# Autodesk Inventor assembly: ASY PRS 9800 DrainSystemBottom_D1200
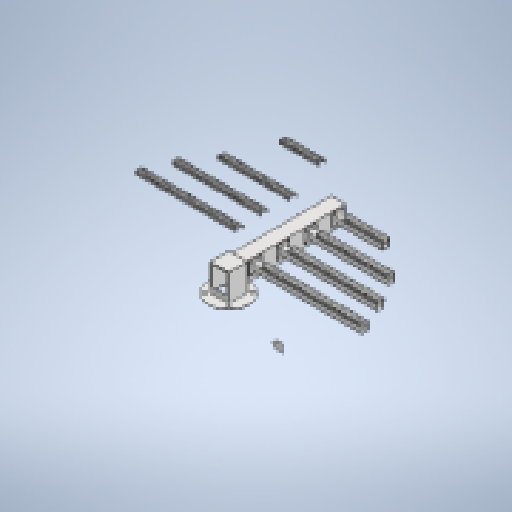
[picture p0: Inventor's stored thumbnail of the model, 512x512]
Saved by Autodesk Inventor 2026.2 (Build 302298000, 298)
## iProperties
Created: 2026-05-12
Part Number: ASY PRS 9800 DrainSystemBottom_D1200
Document SubType Name: Assembly
Designer: admin
Author: admin
## Documents named in this file (22)
- C:\Users\admin\Documents\Inventor\PRS-Purovsk\ASY PRS 9800 DrainSystemBottom_D1200.iam
- C:\Users\admin\Documents\Inventor\PRS-Purovsk\PRS 9651 DrSysB MAIN  FLANGE_D1200.ipt
- C:\Users\admin\Documents\Inventor\PRS-Purovsk\PRS 1425 DrSysB Way FLANGE_D1200.ipt
- C:\Users\admin\Documents\Inventor\PRS-Purovsk\PRS 1401 DrSysB DIMentions_D1200.ipt
- C:\Users\admin\Documents\Inventor\PRS-Purovsk\PRS 1662 DrSysB way tube 4_D1200.ipt
- C:\Users\admin\Documents\Inventor\PRS-Purovsk\PRS 1652 DrSysB Central tube wall_D1200.ipt
- C:\Users\admin\Documents\Inventor\PRS-Purovsk\PRS 1662 DrSysB way tube 2_D1200.ipt
- C:\Users\admin\Documents\Inventor\PRS-Purovsk\PRS 1665 DrSysB CUP 1_D1200.ipt
- C:\Users\admin\Documents\Inventor\PRS-Purovsk\PRS-1666 FDS 1000 CUP 1_D1200.ipt
- C:\Users\admin\Documents\Inventor\PRS-Purovsk\PRS 1422 DrSysB diameter way up_D1200.ipt
- C:\Users\admin\Documents\Inventor\PRS-Purovsk\PRS 1423 DrSysB diameter way down_D1200.ipt
- C:\Users\admin\Documents\Inventor\PRS-Purovsk\PRS 1424 DrSysB diam way cup_D1200.ipt
- C:\Users\admin\Documents\Inventor\PRS-Purovsk\PRS 1661 DrSysB way tube 1_D1200.ipt
- C:\Users\admin\Documents\Inventor\PRS-Purovsk\PRS 5311 DrSysB roof 1_D1200.ipt
- C:\Users\admin\Documents\Inventor\PRS-Purovsk\PRS 5321 DrSysB roof 2_D1200.ipt
- C:\Users\admin\Documents\Inventor\PRS-Purovsk\PRS 5333 DrSysB roof 3_D1200.ipt
- C:\Users\admin\Documents\Inventor\PRS-Purovsk\PRS 1662 DrSysB way tube 44_D1200.ipt
- C:\Users\admin\Documents\Inventor\PRS-Purovsk\PRS 5335 DrSysB roof 33_D1200.ipt
- C:\Users\admin\Documents\Inventor\PRS-Purovsk\PRS 7623 DrSysB  roof 1_1200x7.5_D1200.ipt
- C:\Users\admin\Documents\Inventor\PRS-Purovsk\PRS 5322 DrSysB roof 2_1200x7.5_D1200.ipt
- C:\Users\admin\Documents\Inventor\PRS-Purovsk\PRS 5334 DrSysB roof 3_1200x7.5_D1200.ipt
- C:\Users\admin\Documents\Inventor\PRS-Purovsk\PRS 5336 DrSysB roof 3_44_1200x7.5_D1200.ipt
## Components (28 placed, 21 different names)
1. PRS 9651 DrSysB MAIN  FLANGE_D1200:1 — Flush:8, Flush:7, Mate:3
2. PRS 1425 DrSysB Way FLANGE_D1200:1 — Rigid:4, Rigid:19
3. PRS 1401 DrSysB DIMentions_D1200:1
4. PRS 1662 DrSysB way tube 4_D1200:1 — Flush:5, Mate:9, Mate:7, Rigid:21
5. PRS 1652 DrSysB Central tube wall_D1200:1 — Flush:8, Flush:7, Mate:10, Rigid:24, Rigid:22
6. PRS 1652 DrSysB Central tube wall_D1200:2 — Mate:3, Rigid:22
7. PRS 1662 DrSysB way tube 2_D1200:1 — Mate:8, Flush:6, Mate:6, Rigid:20
8. PRS 1665 DrSysB CUP 1_D1200:1 — Mate:10
9. PRS-1666 FDS 1000 CUP 1_D1200:1
10. PRS 1422 DrSysB diameter way up_D1200:1 — Flush:10, Flush:9, Mate:11, Rigid:23, Rigid:18, Rigid:17, Rigid:16
11. PRS 1423 DrSysB diameter way down_D1200:1 — Rigid:24, Rigid:23, Rigid:4, Rigid:14, Rigid:15, Rigid:13
12. PRS 1424 DrSysB diam way cup_D1200:1 — Flush:10, Flush:9, Mate:11
13. PRS 1425 DrSysB Way FLANGE_D1200:2 — Rigid:20, Rigid:14
14. PRS 1425 DrSysB Way FLANGE_D1200:3 — Rigid:21, Rigid:15
15. PRS 1425 DrSysB Way FLANGE_D1200:4 — Rigid:18
16. PRS 1425 DrSysB Way FLANGE_D1200:5 — Rigid:17
17. PRS 1425 DrSysB Way FLANGE_D1200:6 — Rigid:16
18. PRS 1661 DrSysB way tube 1_D1200:1 — Mate:5, Mate:4, Flush:4, Rigid:19
19. PRS 5311 DrSysB roof 1_D1200:1 — Mate:5, Mate:4, Flush:4
20. PRS 5321 DrSysB roof 2_D1200:1 — Mate:8, Flush:6, Mate:6
21. PRS 5333 DrSysB roof 3_D1200:1 — Flush:5, Mate:9, Mate:7
22. PRS 1662 DrSysB way tube 44_D1200:1 — Mate:12, Mate:13, Flush:9, Rigid:14
23. PRS 5335 DrSysB roof 33_D1200:1 — Mate:12, Mate:13, Flush:9
24. PRS 1425 DrSysB Way FLANGE_D1200:7 — Rigid:13, Rigid:14
25. PRS 7623 DrSysB  roof 1_1200x7.5_D1200:1
26. PRS 5322 DrSysB roof 2_1200x7.5_D1200:1
27. PRS 5334 DrSysB roof 3_1200x7.5_D1200:1
28. PRS 5336 DrSysB roof 3_44_1200x7.5_D1200:1
## Relationships (33: WeldJoint 14, Mate 11, Flush 8)
- Flush:8: PRS 9651 DrSysB MAIN  FLANGE_D1200:1 ↔ PRS 1652 DrSysB Central tube wall_D1200:1
- Flush:7: PRS 9651 DrSysB MAIN  FLANGE_D1200:1 ↔ PRS 1652 DrSysB Central tube wall_D1200:1
- Mate:10: PRS 1652 DrSysB Central tube wall_D1200:1 ↔ PRS 1665 DrSysB CUP 1_D1200:1
- Flush:10 (1 mm): PRS 1422 DrSysB diameter way up_D1200:1 ↔ PRS 1424 DrSysB diam way cup_D1200:1
- Flush:9 (-1 mm): PRS 1422 DrSysB diameter way up_D1200:1 ↔ PRS 1424 DrSysB diam way cup_D1200:1
- Mate:11: PRS 1422 DrSysB diameter way up_D1200:1 ↔ PRS 1424 DrSysB diam way cup_D1200:1
- Mate:3: PRS 9651 DrSysB MAIN  FLANGE_D1200:1 ↔ PRS 1652 DrSysB Central tube wall_D1200:2
- Mate:5 (10 mm): PRS 1661 DrSysB way tube 1_D1200:1 ↔ PRS 5311 DrSysB roof 1_D1200:1
- Mate:4: PRS 1661 DrSysB way tube 1_D1200:1 ↔ PRS 5311 DrSysB roof 1_D1200:1
- Flush:4 (40 mm): PRS 1661 DrSysB way tube 1_D1200:1 ↔ PRS 5311 DrSysB roof 1_D1200:1
- Mate:8: PRS 1662 DrSysB way tube 2_D1200:1 ↔ PRS 5321 DrSysB roof 2_D1200:1
- Flush:6 (-40 mm): PRS 1662 DrSysB way tube 2_D1200:1 ↔ PRS 5321 DrSysB roof 2_D1200:1
- Mate:6 (10 mm): PRS 1662 DrSysB way tube 2_D1200:1 ↔ PRS 5321 DrSysB roof 2_D1200:1
- Flush:5 (-40 mm): PRS 1662 DrSysB way tube 4_D1200:1 ↔ PRS 5333 DrSysB roof 3_D1200:1
- Mate:9: PRS 1662 DrSysB way tube 4_D1200:1 ↔ PRS 5333 DrSysB roof 3_D1200:1
- Mate:7 (10 mm): PRS 1662 DrSysB way tube 4_D1200:1 ↔ PRS 5333 DrSysB roof 3_D1200:1
- Rigid:24 [WeldJoint]: PRS 1652 DrSysB Central tube wall_D1200:1 ↔ PRS 1423 DrSysB diameter way down_D1200:1
- Rigid:23 [WeldJoint]: PRS 1422 DrSysB diameter way up_D1200:1 ↔ PRS 1423 DrSysB diameter way down_D1200:1
- Rigid:4 [WeldJoint]: PRS 1425 DrSysB Way FLANGE_D1200:1 ↔ PRS 1423 DrSysB diameter way down_D1200:1
- Rigid:22 [WeldJoint]: PRS 1652 DrSysB Central tube wall_D1200:1 ↔ PRS 1652 DrSysB Central tube wall_D1200:2
- Rigid:20 [WeldJoint] (-2 mm): PRS 1662 DrSysB way tube 2_D1200:1 ↔ PRS 1425 DrSysB Way FLANGE_D1200:2
- Rigid:14 [WeldJoint]: PRS 1423 DrSysB diameter way down_D1200:1 ↔ PRS 1425 DrSysB Way FLANGE_D1200:2
- Rigid:21 [WeldJoint] (-2 mm): PRS 1662 DrSysB way tube 4_D1200:1 ↔ PRS 1425 DrSysB Way FLANGE_D1200:3
- Rigid:15 [WeldJoint]: PRS 1423 DrSysB diameter way down_D1200:1 ↔ PRS 1425 DrSysB Way FLANGE_D1200:3
- Rigid:18 [WeldJoint]: PRS 1422 DrSysB diameter way up_D1200:1 ↔ PRS 1425 DrSysB Way FLANGE_D1200:4
- Rigid:17 [WeldJoint]: PRS 1422 DrSysB diameter way up_D1200:1 ↔ PRS 1425 DrSysB Way FLANGE_D1200:5
- Rigid:16 [WeldJoint]: PRS 1422 DrSysB diameter way up_D1200:1 ↔ PRS 1425 DrSysB Way FLANGE_D1200:6
- Rigid:19 [WeldJoint] (-2 mm): PRS 1425 DrSysB Way FLANGE_D1200:1 ↔ PRS 1661 DrSysB way tube 1_D1200:1
- Mate:12 (10 mm): PRS 1662 DrSysB way tube 44_D1200:1 ↔ PRS 5335 DrSysB roof 33_D1200:1
- Mate:13: PRS 1662 DrSysB way tube 44_D1200:1 ↔ PRS 5335 DrSysB roof 33_D1200:1
- Flush:9 (-40 mm): PRS 1662 DrSysB way tube 44_D1200:1 ↔ PRS 5335 DrSysB roof 33_D1200:1
- Rigid:13 [WeldJoint]: PRS 1423 DrSysB diameter way down_D1200:1 ↔ PRS 1425 DrSysB Way FLANGE_D1200:7
- Rigid:14 [WeldJoint]: PRS 1662 DrSysB way tube 44_D1200:1 ↔ PRS 1425 DrSysB Way FLANGE_D1200:7
